# Autodesk Inventor assembly: base plate 1
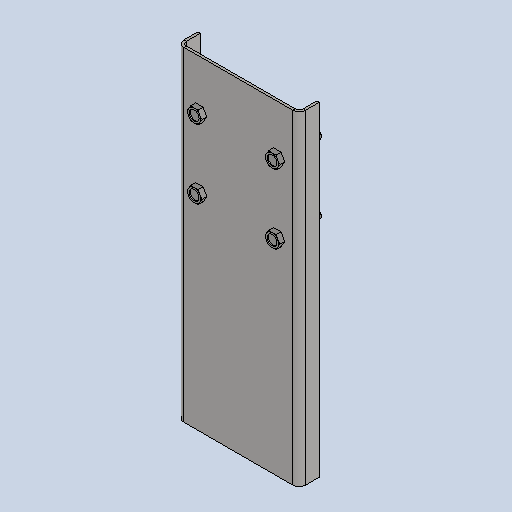
[picture p0: Inventor's stored thumbnail of the model, 512x512]
Saved by Autodesk Inventor 2025 (Build 290162010, 162A)
## iProperties
Created: 2024-04-16
Part Number: base plate 1
Document SubType Name: Assembly
Designer: pokla
Stock Number: базовая пластина
Author: pokla
## Documents named in this file (4)
- C:\Users\admin\YandexDisk-badmisterfox\домашниий пк\Inventor\tale tales\Gusev_Meshalka\ASY Мешалка\Корпус.iam
- C:\Users\admin\YandexDisk-badmisterfox\домашниий пк\Inventor\tale tales\Gusev_Meshalka\ASY Мешалка\Крепление.ipt
- C:\Users\admin\YandexDisk-badmisterfox\домашниий пк\Inventor\tale tales\Gusev_Meshalka\ASY Мешалка\Параметры.ipt
- C:\Users\admin\YandexDisk-badmisterfox\домашниий пк\Inventor\tale tales\Gusev_Meshalka\ASY Мешалка\CSN EN 24015 - M10x50.ipt
## Components (6 placed, 3 different names)
1. Крепление.ipt:1 — Flush:1, Mate:1, Insert:1
2. Параметры.ipt:1
3. CSN EN 24015 - M10x50.ipt:1 — Insert:1
4. CSN EN 24015 - M10x50.ipt:2
5. CSN EN 24015 - M10x50.ipt:3
6. CSN EN 24015 - M10x50.ipt:4
## Component patterns: (4 elements, first: CSN EN 24015 - M10x50.ipt:1)
## Relationships (3: Flush 1, Mate 1, Insert 1)
- Flush:1: Крепление.ipt:1
- Mate:1: Крепление.ipt:1
- Insert:1: Крепление.ipt:1 ↔ CSN EN 24015 - M10x50.ipt:1
